# Autodesk Inventor assembly: minibot
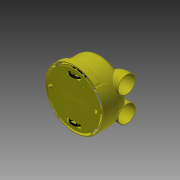
[picture p0: Inventor's stored thumbnail of the model, 180x180]
Saved by Autodesk Inventor 2015 (Build 190159000, 159)
## iProperties
Created: 2015-03-14
Part Number: minibot
Document SubType Name: Assembly
Designer: david_000
Author: david_000
## Documents named in this file (12)
- C:\Users\david_000\Desktop\minibot-code\mechanics\minibot.iam
- C:\Users\david_000\Desktop\minibot-code\mechanics\37D.ipt
- C:\Users\david_000\Desktop\minibot-code\mechanics\Universal Mounting.ipt
- C:\Users\david_000\Desktop\minibot-code\mechanics\80x10.ipt
- C:\Users\david_000\Desktop\minibot-code\mechanics\ArduinoMega2560R3.iam
- C:\Users\david_000\Desktop\minibot-code\mechanics\proteccion_lateral.ipt
- C:\Users\david_000\Desktop\minibot-code\mechanics\base.iam
- C:\Users\david_000\Desktop\minibot-code\mechanics\proteccion_lateral_delantera.ipt
- C:\Users\david_000\Desktop\minibot-code\mechanics\eye.ipt
- C:\Users\david_000\Desktop\minibot-code\mechanics\tapa.ipt
- C:\Users\david_000\Desktop\minibot-code\mechanics\keypad.iam
- C:\Users\david_000\Desktop\minibot-code\mechanics\cupula_partes_2.iam
## Components (17 placed, 11 different names)
1. 37D:1 — Nivelación:2, Coincidencia:14, Coincidencia:21, Coincidencia:22, Coincidencia:23
2. 37D:2 — Coincidencia:13, Nivelación:1, Coincidencia:18, Coincidencia:19, Coincidencia:20
3. Universal Mounting:1 — Coincidencia:7, Coincidencia:8, Coincidencia:9, Nivelación:2, Coincidencia:14
4. 80x10:1 — Coincidencia:7, Coincidencia:8, Coincidencia:9
5. Universal Mounting:2 — Coincidencia:13, Nivelación:1
6. 80x10:2
7. ArduinoMega2560R3:1 [sub-assembly] — Coincidencia:35, Coincidencia:36
8. proteccion_lateral:1 — Coincidencia:15, Coincidencia:16, Coincidencia:17
9. proteccion_lateral:2 — Nivelación:5, Coincidencia:28, Coincidencia:29
10. proteccion_lateral:3 — Nivelación:4, Coincidencia:24, Coincidencia:25
11. base:1 [sub-assembly] — Coincidencia:15, Coincidencia:16, Coincidencia:17, Coincidencia:18, Coincidencia:19, Coincidencia:20, Coincidencia:21, Coincidencia:22, Coincidencia:23, Nivelación:4, Nivelación:5, Coincidencia:24, Coincidencia:25, Coincidencia:28, Coincidencia:29, Coincidencia:31, Coincidencia:32, Coincidencia:33, Coincidencia:35, Coincidencia:36, Coincidencia:42, Coincidencia:43, Coincidencia:44
12. proteccion_lateral_delantera:1 — Coincidencia:31, Coincidencia:32, Coincidencia:33
13. eye:3
14. eye:4
15. tapa:1 — Coincidencia:39, Coincidencia:40, Coincidencia:41
16. keypad:1 [sub-assembly] — Coincidencia:39, Coincidencia:40, Coincidencia:41
17. cupula_partes_2:1 [sub-assembly] — Coincidencia:42, Coincidencia:43, Coincidencia:44
## Relationships (36: Mate 32, Flush 4)
- Coincidencia:7 [Mate]: Universal Mounting:1 ↔ 80x10:1
- Coincidencia:8 [Mate]: Universal Mounting:1 ↔ 80x10:1
- Coincidencia:9 [Mate]: Universal Mounting:1 ↔ 80x10:1
- [Mate]: Universal Mounting:2 ↔ 80x10:2
- [Mate]: Universal Mounting:2 ↔ 80x10:2
- [Mate]: Universal Mounting:2 ↔ 80x10:2
- Coincidencia:13 [Mate]: 37D:2 ↔ Universal Mounting:2
- Nivelación:1 [Flush]: 37D:2 ↔ Universal Mounting:2
- Nivelación:2 [Flush]: 37D:1 ↔ Universal Mounting:1
- Coincidencia:14 [Mate]: 37D:1 ↔ Universal Mounting:1
- Coincidencia:15 [Mate]: proteccion_lateral:1 ↔ base:1
- Coincidencia:16 [Mate]: proteccion_lateral:1 ↔ base:1
- Coincidencia:17 [Mate]: proteccion_lateral:1 ↔ base:1
- Coincidencia:18 [Mate]: 37D:2 ↔ base:1
- Coincidencia:19 [Mate]: 37D:2 ↔ base:1
- Coincidencia:20 [Mate]: 37D:2 ↔ base:1
- Coincidencia:21 [Mate]: 37D:1 ↔ base:1
- Coincidencia:22 [Mate]: 37D:1 ↔ base:1
- Coincidencia:23 [Mate]: 37D:1 ↔ base:1
- Nivelación:4 [Flush]: proteccion_lateral:3 ↔ base:1
- Nivelación:5 [Flush]: proteccion_lateral:2 ↔ base:1
- Coincidencia:24 [Mate]: proteccion_lateral:3 ↔ base:1
- Coincidencia:25 [Mate]: proteccion_lateral:3 ↔ base:1
- Coincidencia:28 [Mate]: proteccion_lateral:2 ↔ base:1
- Coincidencia:29 [Mate]: proteccion_lateral:2 ↔ base:1
- Coincidencia:31 [Mate]: base:1 ↔ proteccion_lateral_delantera:1
- Coincidencia:32 [Mate]: base:1 ↔ proteccion_lateral_delantera:1
- Coincidencia:33 [Mate]: base:1 ↔ proteccion_lateral_delantera:1
- Coincidencia:35 [Mate] (10 mm): ArduinoMega2560R3:1 ↔ base:1
- Coincidencia:36 [Mate] (5 mm): ArduinoMega2560R3:1 ↔ base:1
- Coincidencia:39 [Mate]: tapa:1 ↔ keypad:1
- Coincidencia:40 [Mate]: tapa:1 ↔ keypad:1
- Coincidencia:41 [Mate]: tapa:1 ↔ keypad:1
- Coincidencia:42 [Mate]: base:1 ↔ cupula_partes_2:1
- Coincidencia:43 [Mate]: base:1 ↔ cupula_partes_2:1
- Coincidencia:44 [Mate]: base:1 ↔ cupula_partes_2:1
## Named parameters: d9_d6 = 0 mm, d10_d7 = 0 mm, d11_d8 = 0 mm
